# Autodesk Inventor assembly: LedCube
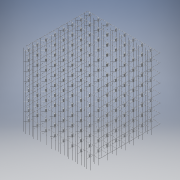
[picture p0: Inventor's stored thumbnail of the model, 180x180]
Saved by Autodesk Inventor 2019.3 (Build 233278000, 278)
## iProperties
Created: 2019-01-10
Part Number: LedCube
Material: Generisch
Document SubType Name: Assembly
Designer: Jonas
Author: Jonas
## Documents named in this file (3)
- C:\Users\Jonas\Desktop\RGBCube\RGBCubev2\CAD\Led\LedCube.iam
- C:\Users\Jonas\Desktop\RGBCube\RGBCubev2\CAD\Led\LedPlane.iam
- C:\Users\Jonas\Desktop\RGBCube\RGBCubev2\CAD\Led\WireCathode2.ipt
## Components (24 placed, 2 different names)
1. LedPlane:1 [sub-assembly] — Passend:58, Passend:59, Passend:60, Passend:63, Passend:65, Passend:66, Passend:69, Tangential:2, Tangential:3, Tangential:6, Tangential:8, Tangential:10, Tangential:12, Tangential:14, Tangential:16, Tangential:18, Tangential:20, Tangential:22, Tangential:24, Tangential:26, Tangential:28, Tangential:30, Tangential:32
2. LedPlane:2 [sub-assembly] — Passend:56, Passend:57, Passend:61, Passend:62, Passend:64, Passend:67, Passend:68
3. LedPlane:3 [sub-assembly] — Passend:13, Passend:14, Passend:15, Passend:16, Passend:17, Passend:18, Passend:19, Passend:55
4. LedPlane:4 [sub-assembly] — Passend:20, Passend:21, Passend:24, Passend:25, Passend:30, Passend:54
5. LedPlane:5 [sub-assembly] — Passend:22, Passend:23, Passend:26, Passend:27, Passend:31, Passend:53
6. LedPlane:6 [sub-assembly] — Passend:32, Passend:33, Passend:38, Passend:39, Passend:44, Passend:47, Passend:52
7. LedPlane:7 [sub-assembly] — Passend:34, Passend:35, Passend:40, Passend:41, Passend:45, Passend:48, Passend:51
8. LedPlane:8 [sub-assembly] — Passend:36, Passend:37, Passend:42, Passend:43, Passend:46, Passend:49, Passend:50, Winkel:1, Tangential:1, Tangential:4, Tangential:5, Tangential:7, Tangential:9, Tangential:11, Tangential:13, Tangential:15, Tangential:17, Tangential:19, Tangential:21, Tangential:23, Tangential:25, Tangential:27, Tangential:29, Tangential:31
9. WireCathode2:1 — Winkel:1, Tangential:1, Tangential:2, Passend:70, Passend:71
10. WireCathode2:2 — Passend:72, Passend:73, Tangential:3, Tangential:4
11. WireCathode2:3 — Passend:74, Tangential:5, Tangential:6, Passend:75
12. WireCathode2:4 — Passend:76, Tangential:7, Passend:77, Tangential:8
13. WireCathode2:5 — Passend:78, Tangential:9, Tangential:10, Passend:79
14. WireCathode2:6 — Passend:80, Tangential:11, Tangential:12, Passend:81
15. WireCathode2:7 — Passend:82, Tangential:13, Tangential:14, Passend:83
16. WireCathode2:8 — Passend:84, Tangential:15, Tangential:16, Passend:85
17. WireCathode2:9 — Passend:86, Tangential:17, Tangential:18, Passend:87
18. WireCathode2:10 — Passend:88, Tangential:19, Passend:89, Tangential:20
19. WireCathode2:11 — Passend:90, Tangential:21, Tangential:22, Passend:91
20. WireCathode2:12 — Passend:92, Tangential:23, Tangential:24, Passend:93
21. WireCathode2:13 — Passend:94, Tangential:25, Tangential:26, Passend:95
22. WireCathode2:14 — Passend:96, Tangential:27, Tangential:28, Passend:97
23. WireCathode2:15 — Passend:98, Tangential:29, Tangential:30, Passend:99
24. WireCathode2:16 — Tangential:31, Tangential:32, Passend:100, Passend:101
## Relationships (123: Mate 87, Tangent 32, Flush 3, Angle 1)
- Fluchtend:1 [Flush] (-250 mm)
- Passend:13 [Mate]: LedPlane:3
- Passend:14 [Mate]: LedPlane:3
- Passend:15 [Mate] (60 mm): LedPlane:3
- Passend:16 [Mate]: LedPlane:3
- Passend:17 [Mate]: LedPlane:3
- Passend:18 [Mate] (60 mm): LedPlane:3
- Passend:19 [Mate] (60 mm): LedPlane:3
- Passend:20 [Mate]: LedPlane:4
- Passend:21 [Mate]: LedPlane:4
- Passend:22 [Mate]: LedPlane:5
- Passend:23 [Mate]: LedPlane:5
- Passend:24 [Mate]: LedPlane:4
- Passend:25 [Mate]: LedPlane:4
- Passend:26 [Mate]: LedPlane:5
- Passend:27 [Mate]: LedPlane:5
- Passend:30 [Mate] (90 mm): LedPlane:4
- Passend:31 [Mate] (120 mm): LedPlane:5
- Passend:32 [Mate]: LedPlane:6
- Passend:33 [Mate]: LedPlane:6
- Passend:34 [Mate]: LedPlane:7
- Passend:35 [Mate]: LedPlane:7
- Passend:36 [Mate]: LedPlane:8
- Passend:37 [Mate]: LedPlane:8
- Passend:38 [Mate]: LedPlane:6
- Passend:39 [Mate]: LedPlane:6
- Passend:40 [Mate]: LedPlane:7
- Passend:41 [Mate]: LedPlane:7
- Passend:42 [Mate]: LedPlane:8
- Passend:43 [Mate]: LedPlane:8
- Passend:44 [Mate] (150 mm): LedPlane:6
- Passend:45 [Mate] (180 mm): LedPlane:7
- Passend:46 [Mate] (210 mm): LedPlane:8
- Passend:47 [Mate] (150 mm): LedPlane:6
- Passend:48 [Mate] (180 mm): LedPlane:7
- Passend:49 [Mate] (210 mm): LedPlane:8
- Passend:50 [Mate]: LedPlane:8
- Passend:51 [Mate]: LedPlane:7
- Passend:52 [Mate]: LedPlane:6
- Passend:53 [Mate]: LedPlane:5
- Passend:54 [Mate]: LedPlane:4
- Passend:55 [Mate]: LedPlane:3
- Passend:56 [Mate]: LedPlane:2
- Passend:57 [Mate]: LedPlane:2
- Passend:58 [Mate]: LedPlane:1
- Passend:59 [Mate]: LedPlane:1
- Passend:60 [Mate]: LedPlane:1
- Passend:61 [Mate]: LedPlane:2
- Passend:62 [Mate]: LedPlane:2
- Passend:63 [Mate]: LedPlane:1
- Passend:64 [Mate] (30 mm): LedPlane:2
- Passend:65 [Mate]: LedPlane:1
- Passend:66 [Mate]: LedPlane:1
- Passend:67 [Mate] (30 mm): LedPlane:2
- Passend:68 [Mate]: LedPlane:2
- Passend:69 [Mate]: LedPlane:1
- Winkel:1 [Angle] (-90 deg): LedPlane:8 ↔ WireCathode2:1
- Tangential:1: LedPlane:8 ↔ WireCathode2:1
- Tangential:2: LedPlane:1 ↔ WireCathode2:1
- Passend:70 [Mate]: WireCathode2:1
- Passend:71 [Mate]: WireCathode2:1
- Passend:72 [Mate]: WireCathode2:2
- Passend:73 [Mate]: WireCathode2:2
- Tangential:3: LedPlane:1 ↔ WireCathode2:2
- Tangential:4: LedPlane:8 ↔ WireCathode2:2
- Passend:74 [Mate]: WireCathode2:3
- Tangential:5: LedPlane:8 ↔ WireCathode2:3
- Tangential:6: LedPlane:1 ↔ WireCathode2:3
- Passend:75 [Mate]: WireCathode2:3
- Passend:76 [Mate]: WireCathode2:4
- Tangential:7: LedPlane:8 ↔ WireCathode2:4
- Passend:77 [Mate]: WireCathode2:4
- Tangential:8: LedPlane:1 ↔ WireCathode2:4
- Passend:78 [Mate]: WireCathode2:5
- Tangential:9: LedPlane:8 ↔ WireCathode2:5
- Tangential:10: LedPlane:1 ↔ WireCathode2:5
- Passend:79 [Mate]: WireCathode2:5
- Passend:80 [Mate]: WireCathode2:6
- Tangential:11: LedPlane:8 ↔ WireCathode2:6
- Tangential:12: LedPlane:1 ↔ WireCathode2:6
- Passend:81 [Mate]: WireCathode2:6
- Passend:82 [Mate]: WireCathode2:7
- Tangential:13: LedPlane:8 ↔ WireCathode2:7
- Tangential:14: LedPlane:1 ↔ WireCathode2:7
- Passend:83 [Mate]: WireCathode2:7
- Passend:84 [Mate]: WireCathode2:8
- Tangential:15: LedPlane:8 ↔ WireCathode2:8
- Tangential:16: LedPlane:1 ↔ WireCathode2:8
- Passend:85 [Mate]: WireCathode2:8
- Passend:86 [Mate]: WireCathode2:9
- Tangential:17: LedPlane:8 ↔ WireCathode2:9
- Tangential:18: LedPlane:1 ↔ WireCathode2:9
- Passend:87 [Mate]: WireCathode2:9
- Passend:88 [Mate]: WireCathode2:10
- Tangential:19: LedPlane:8 ↔ WireCathode2:10
- Passend:89 [Mate]: WireCathode2:10
- Tangential:20: LedPlane:1 ↔ WireCathode2:10
- Passend:90 [Mate]: WireCathode2:11
- Tangential:21: LedPlane:8 ↔ WireCathode2:11
- Tangential:22: LedPlane:1 ↔ WireCathode2:11
- Passend:91 [Mate]: WireCathode2:11
- Passend:92 [Mate]: WireCathode2:12
- Tangential:23: LedPlane:8 ↔ WireCathode2:12
- Tangential:24: LedPlane:1 ↔ WireCathode2:12
- Passend:93 [Mate]: WireCathode2:12
- Passend:94 [Mate]: WireCathode2:13
- Tangential:25: LedPlane:8 ↔ WireCathode2:13
- Tangential:26: LedPlane:1 ↔ WireCathode2:13
- Passend:95 [Mate]: WireCathode2:13
- Passend:96 [Mate]: WireCathode2:14
- Tangential:27: LedPlane:8 ↔ WireCathode2:14
- Tangential:28: LedPlane:1 ↔ WireCathode2:14
- Passend:97 [Mate]: WireCathode2:14
- Passend:98 [Mate]: WireCathode2:15
- Tangential:29: LedPlane:8 ↔ WireCathode2:15
- Tangential:30: LedPlane:1 ↔ WireCathode2:15
- Passend:99 [Mate]: WireCathode2:15
- Tangential:31: LedPlane:8 ↔ WireCathode2:16
- Tangential:32: LedPlane:1 ↔ WireCathode2:16
- Passend:100 [Mate]: WireCathode2:16
- Passend:101 [Mate]: WireCathode2:16
- Fluchtend:2 [Flush] (210 mm)
- Fluchtend:3 [Flush] (-23 mm)
